# Autodesk Inventor assembly: TEST_STACK_V1
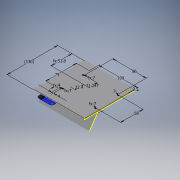
[picture p0: Inventor's stored thumbnail of the model, 180x180]
Saved by Autodesk Inventor 2019 (Build 230136000, 136)
## iProperties
Created: 2020-02-13
Part Number: TEST_STACK_V1
Document SubType Name: Assembly
Designer: close
Author: close
## Documents named in this file (4)
- C:\Users\close\Desktop\CAD BARC-ROAR\Enclosure\V_1\TEST_STACK_V1.iam
- C:\Users\close\Desktop\CAD BARC-ROAR\Enclosure\V_1\angle test.ipt
- C:\Users\close\Desktop\CAD BARC-ROAR\Dependencies\Nvidia Jetson Nano\P3450_P3449_A02_P3448_A02.iam
- C:\Users\close\Desktop\CAD BARC-ROAR\Dependencies\Splitter Board\SplitterBoard.iam
## Components (3 placed, 3 different names)
1. angle test:1
2. P3450_P3449_A02_P3448_A02:1 [sub-assembly] — Mate:1
3. SplitterBoard:1 [sub-assembly] — Mate:1
## Relationships (1: Mate 1)
- Mate:1 (-15 mm): P3450_P3449_A02_P3448_A02:1 ↔ SplitterBoard:1
